# Autodesk Inventor assembly: MX-106_with_horn_MIR_MIR
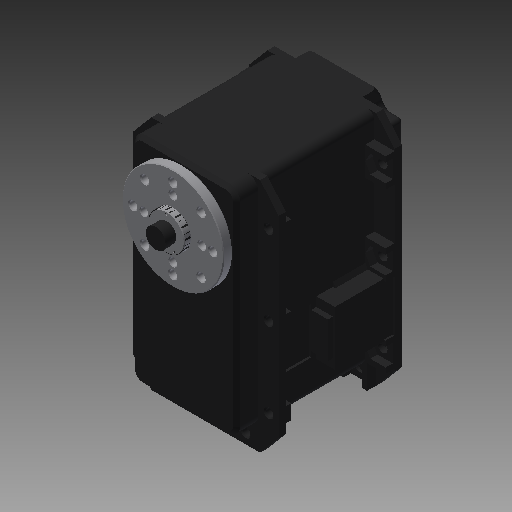
[picture p0: Inventor's stored thumbnail of the model, 512x512]
Saved by Autodesk Inventor 2018 (Build 220112000, 112)
## iProperties
Created: 2015-05-09
Part Number: MX-106_with_horn_MIR_MIR
Document SubType Name: Assembly
Designer: bitbots
Mass: 86.5149 g
Surface Area: 177.097 cm^2
Volume: 86.5149 cm^3
Density: 1 g/cm^3
Author: bitbots
## Documents named in this file (3)
- C:\Users\bitbots\Desktop\bitbots_hardware\wolfgang\assembly\motors\MX106\MX-106_with_horn_MIR_MIR.iam
- C:\Users\bitbots\Desktop\bitbots_hardware\wolfgang\assembly\motors\MX106\MX-106_MIR_MIR.ipt
- C:\Users\bitbots\Desktop\bitbots_hardware\wolfgang\assembly\motors\MX64\HN05-N101_MIR1_MIR.ipt
## Components (2 placed, 2 different names)
1. MX-106_MIR_MIR:1 — Rotational:1
2. HN05-N101_MIR1_MIR:1 — Rotational:1
## Relationships (1: RevoluteJoint 1)
- Rotational:1 [RevoluteJoint] (-7 mm): MX-106_MIR_MIR:1 ↔ HN05-N101_MIR1_MIR:1
